# Autodesk Inventor assembly: Assembly1
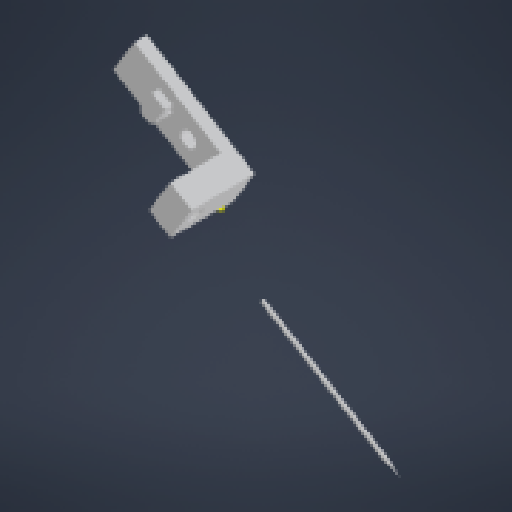
[picture p0: Inventor's stored thumbnail of the model, 512x512]
Saved by Autodesk Inventor 2026 (Build 300175050, 175E)
## iProperties
Created: 2025-06-30
Part Number: Assembly1
Document SubType Name: Assembly
Designer: Tobymegacat
Author: Tobymegacat
## Documents named in this file (4)
- C:\Users\herve\OneDrive\桌面\NIST\Inventor\Assembly1.iam
- C:\Users\herve\OneDrive\桌面\NIST\Inventor\Upper probe arm.ipt
- C:\Users\herve\OneDrive\桌面\NIST\Inventor\fake m3 screw.ipt
- C:\Users\herve\OneDrive\桌面\NIST\Inventor\fake needle.ipt
## Components (3 placed, 3 different names)
1. Upper probe arm:1 — Cylindrical:1
2. fake m3 screw:1 — Cylindrical:1, Rigid:1
3. fake needle:1 — Rigid:1
## Relationships (2: CylindricalJoint 1, WeldJoint 1)
- Cylindrical:1: Upper probe arm:1 ↔ fake m3 screw:1
- Rigid:1 [WeldJoint]: fake m3 screw:1 ↔ fake needle:1
